# Autodesk Inventor assembly: 基本構造
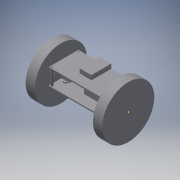
[picture p0: Inventor's stored thumbnail of the model, 180x180]
Saved by Autodesk Inventor 2017 (Build 210142000, 142)
## iProperties
Part Number: 基本構造
Material: 一般
Document SubType Name: Assembly
Designer: HISAAKI
Author: HISAAKI
## Documents named in this file (10)
- C:\Users\HISAAKI\Documents\LYNCS\CanSat\2017種子島\cansat-structure\基本構造.iam
- C:\Users\HISAAKI\Documents\LYNCS\CanSat\2017種子島\cansat-structure\基本板.ipt
- C:\Users\HISAAKI\Documents\LYNCS\CanSat\2017種子島\cansat-structure\既成部品\ブラケット.ipt
- C:\Users\HISAAKI\Documents\LYNCS\CanSat\2017種子島\cansat-structure\既成部品\モータ.ipt
- C:\Users\HISAAKI\Documents\LYNCS\CanSat\2017種子島\cansat-structure\ハブver1.1.ipt
- C:\Users\HISAAKI\Documents\LYNCS\CanSat\2017種子島\cansat-structure\タイヤスポンジ部分.ipt
- C:\Users\HISAAKI\Documents\LYNCS\CanSat\2017種子島\cansat-structure\既成部品\リポ電池.ipt
- C:\Users\HISAAKI\Documents\LYNCS\CanSat\2017種子島\cansat-structure\基本板上.ipt
- C:\Users\HISAAKI\Documents\LYNCS\CanSat\2017種子島\cansat-structure\既成部品\mbed.ipt
- C:\Users\HISAAKI\Documents\LYNCS\CanSat\2017種子島\cansat-structure\既成部品\スペーサ.ipt
## Components (16 placed, 9 different names)
1. 基本板:1 — メイト:1, メイト:2, メイト:3, メイト:4, メイト:5, メイト:6, フラッシュ:1, フラッシュ:2, メイト:19, メイト:20, メイト:21, メイト:23, メイト:24, メイト:25, メイト:26, メイト:27, メイト:28, メイト:29, メイト:30
2. ブラケット:1 — メイト:1, メイト:2, メイト:6, メイト:9, メイト:10
3. ブラケット:2 — メイト:3, メイト:4, メイト:5, メイト:7, メイト:8
4. モータ:1 — フラッシュ:2, メイト:9, メイト:10, メイト:13, メイト:14
5. モータ:2 — フラッシュ:1, メイト:7, メイト:8, メイト:11, メイト:12
6. ハブver1.1:1 — メイト:11, メイト:12, メイト:17, メイト:18
7. ハブver1.1:2 — メイト:13, メイト:14, メイト:15, メイト:16
8. タイヤスポンジ部分:1 — メイト:15, メイト:16
9. タイヤスポンジ部分:2 — メイト:17, メイト:18
10. リポ電池:1 — メイト:19
11. 基本板上:1 — メイト:20, メイト:21, メイト:22, フラッシュ:3, メイト:31
12. mbed:1 — メイト:22, フラッシュ:3
13. スペーサ:1 — メイト:23, メイト:29
14. スペーサ:2 — メイト:25, メイト:28
15. スペーサ:3 — メイト:24, メイト:30, メイト:31
16. スペーサ:4 — メイト:26, メイト:27
## Relationships (34: Mate 31, Flush 3)
- メイト:1 [Mate]: 基本板:1 ↔ ブラケット:1
- メイト:2 [Mate]: 基本板:1 ↔ ブラケット:1
- メイト:3 [Mate]: 基本板:1 ↔ ブラケット:2
- メイト:4 [Mate]: 基本板:1 ↔ ブラケット:2
- メイト:5 [Mate]: 基本板:1 ↔ ブラケット:2
- メイト:6 [Mate]: 基本板:1 ↔ ブラケット:1
- フラッシュ:1 [Flush]: 基本板:1 ↔ モータ:2
- メイト:7 [Mate]: ブラケット:2 ↔ モータ:2
- メイト:8 [Mate]: ブラケット:2 ↔ モータ:2
- フラッシュ:2 [Flush]: 基本板:1 ↔ モータ:1
- メイト:9 [Mate]: ブラケット:1 ↔ モータ:1
- メイト:10 [Mate]: ブラケット:1 ↔ モータ:1
- メイト:11 [Mate]: モータ:2 ↔ ハブver1.1:1
- メイト:12 [Mate]: モータ:2 ↔ ハブver1.1:1
- メイト:13 [Mate]: モータ:1 ↔ ハブver1.1:2
- メイト:14 [Mate]: モータ:1 ↔ ハブver1.1:2
- メイト:15 [Mate]: ハブver1.1:2 ↔ タイヤスポンジ部分:1
- メイト:16 [Mate]: ハブver1.1:2 ↔ タイヤスポンジ部分:1
- メイト:17 [Mate]: ハブver1.1:1 ↔ タイヤスポンジ部分:2
- メイト:18 [Mate]: ハブver1.1:1 ↔ タイヤスポンジ部分:2
- メイト:19 [Mate]: 基本板:1 ↔ リポ電池:1
- メイト:20 [Mate]: 基本板:1 ↔ 基本板上:1
- メイト:21 [Mate]: 基本板:1 ↔ 基本板上:1
- メイト:22 [Mate]: 基本板上:1 ↔ mbed:1
- フラッシュ:3 [Flush]: 基本板上:1 ↔ mbed:1
- メイト:23 [Mate]: 基本板:1 ↔ スペーサ:1
- メイト:24 [Mate]: 基本板:1 ↔ スペーサ:3
- メイト:25 [Mate]: 基本板:1 ↔ スペーサ:2
- メイト:26 [Mate]: 基本板:1 ↔ スペーサ:4
- メイト:27 [Mate]: 基本板:1 ↔ スペーサ:4
- メイト:28 [Mate]: 基本板:1 ↔ スペーサ:2
- メイト:29 [Mate]: 基本板:1 ↔ スペーサ:1
- メイト:30 [Mate]: 基本板:1 ↔ スペーサ:3
- メイト:31 [Mate]: 基本板上:1 ↔ スペーサ:3
